# Autodesk Inventor assembly: Shooter Assembly v2
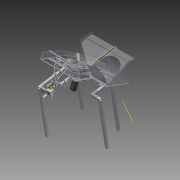
[picture p0: Inventor's stored thumbnail of the model, 180x180]
Saved by Autodesk Inventor 2013 (Build 170138000, 138)
## iProperties
Created: 2013-01-15
Part Number: Shooter Assembly v2
Document SubType Name: Assembly
Designer: actoennies
Mass: 9287.46 g
Surface Area: 30291.7 cm^2
Volume: 4988.3 cm^3
Density: 1.86185 g/cm^3
Author: actoennies
## Documents named in this file (40)
- H:\frc2013CAD-master\Launcher\Shooter\Shooter Assembly v2.iam
- H:\frc2013CAD-master\Launcher\Shooter\Bearing Mount v1.ipt
- H:\frc2013CAD-master\Launcher\Shooter\Outer Rail v1.ipt
- H:\frc2013CAD-master\Launcher\Shooter\Runner Rails v2.ipt
- H:\frc2013CAD-master\Launcher\Shooter\Bearing.ipt
- H:\frc2013CAD-master\Launcher\Shooter\Flywheel Assembly.iam
- H:\frc2013CAD-master\Launcher\Shooter\Shooter Mounter.ipt
- H:\frc2013CAD-master\Launcher\Shooter\Bearing Mount 2 v1.ipt
- H:\frc2013CAD-master\Launcher\Shooter\Shorter Shaft.ipt
- H:\frc2013CAD-master\Launcher\Shooter\Spacer Rube.ipt
- H:\frc2013CAD-master\Launcher\Shooter\Edge Mount.ipt
- H:\frc2013CAD-master\Launcher\Shooter\Square Tube.ipt
- H:\frc2013CAD-master\Launcher\Shooter\Flange Bearing Mount Tower.ipt
- H:\frc2013CAD-master\Launcher\Shooter\Flange Bearing Mount Tower Mirror.ipt
- H:\frc2013CAD-master\Launcher\Shooter\Bearing Mount Top.ipt
- H:\frc2013CAD-master\Launcher\Shooter\Square Motor Mount.ipt
- H:\frc2013CAD-master\Launcher\Shooter\Shooter Assembly v2\Design Accelerator\Spur Gears1.iam
- H:\frc2013CAD-master\Launcher\Parts\Imported Components\Snow Blower Motor\Snow Blower Motor.iam
- H:\frc2013CAD-master\Launcher\Shooter\Snowblower Motor Mount.ipt
- H:\frc2013CAD-master\Launcher\Shooter\8mm shaft.ipt
- H:\frc2013CAD-master\Launcher\Shooter\CIM Bearing.ipt
- H:\frc2013CAD-master\Launcher\Parts\8 Plaction Wheel.iam
- H:\frc2013CAD-master\Launcher\Shooter\Square Tube 2.ipt
- H:\frc2013CAD-master\Launcher\Parts\CIM Motor\Motors_FR801-001.iam
- H:\frc2013CAD-master\Launcher\Shooter\Cim Mount.ipt
- H:\frc2013CAD-master\Launcher\Shooter\Hub v1.ipt
- H:\frc2013CAD-master\Launcher\Shooter\Camera Traffic Light Mount.ipt
- H:\frc2013CAD-master\Launcher\Shooter\Camera Gusset Plat.ipt
- H:\frc2013CAD-master\Launcher\Shooter\Square Tube 3.ipt
- H:\frc2013CAD-master\Launcher\Shooter\edge mount shortened.ipt
- H:\frc2013CAD-master\Launcher\Shooter\Camera.ipt
- H:\frc2013CAD-master\Launcher\Shooter\Square Tube 6.ipt
- H:\frc2013CAD-master\Launcher\Parts\NR-025_5-D(F,D-770).iam
- H:\frc2013CAD-master\Launcher\Shooter\Cylinder Mount.ipt
- H:\frc2013CAD-master\Launcher\Shooter\Cylinder Mount 2.ipt
- H:\frc2013CAD-master\Launcher\Shooter\Gusset Connector.ipt
- H:\frc2013CAD-master\Launcher\Shooter\Gusset Connector 2.ipt
- H:\frc2013CAD-master\Launcher\Shooter\Upper Rails.ipt
- H:\frc2013CAD-master\Launcher\Hopper New\Hopper Assembly.iam
- H:\frc2013CAD-master\Launcher\Hopper New\Puller Mechanism.ipt
## Components (52 placed, 39 different names)
1. Bearing Mount v1:1 — Insert:13, Insert:26, Insert:27, Mate:62, Mate:63, Flush:70, Insert:60, Insert:61, Mate:167
2. Outer Rail v1:1 — Insert:13, Insert:47, Insert:48, Flush:70, Mate:165
3. Runner Rails v2:1 — Insert:60, Insert:61, Mate:166
4. Flywheel Assembly:1 [sub-assembly] — Mate:61, Flush:30, Mate:68, Flush:31
5. Shooter Mounter:1 — Insert:26, Insert:27, Insert:34, Flush:11, Insert:35, Insert:36, Insert:37, Insert:38, Flush:19, Mate:45, Flush:40, Flush:61, Flush:62, Flush:63, Flush:64, Mate:154, Mate:155, Mate:156, Mate:157, Flush:65, Flush:72, Angle:6, Angle:7
6. Spacer Rube:1 — Insert:34, Flush:11
7. Bearing Mount 2 v1:1 — Insert:37, Insert:38, Insert:40
8. Bearing Mount 2 v1:2 — Insert:35, Insert:36, Insert:39
9. Bearing:3 — Insert:40, Flush:13, Mate:14, Mate:15
10. Bearing:4 — Insert:39, Flush:12, Mate:12, Mate:13, Mate:36, Mate:44
11. Shorter Shaft:1 — Flush:12, Mate:12, Mate:13, Mate:37
12. Shorter Shaft:2 — Flush:13, Mate:14, Mate:15, Mate:38
13. Edge Mount:2 — Flush:34, Mate:104, Flush:48, Mate:105, Mate:106, Flush:51, Flush:52, Flush:68
14. Square Tube:2 — Insert:41, Insert:42, Flush:19, Flush:23, Mate:52, Flush:27, Mate:81, Flush:32, Mate:93, Flush:41, Flush:42, Mate:125, Mate:126, Mate:130, Flush:50
15. Flange Bearing Mount Tower:1 — Insert:41, Insert:42, Insert:43
16. Bearing:5 — Insert:43, Mate:36, Mate:37
17. Flange Bearing Mount Tower Mirror:1 — Flush:55, Flush:56, Mate:135, Insert:59
18. Bearing:6 — Mate:38, Insert:59
19. Bearing Mount Top:1 — Insert:47, Insert:48, Mate:65, Mate:66, Mate:68, Mate:162, Mate:163, Mate:164
20. Square Motor Mount:1 — Flush:23, Mate:47, Mate:51, Flush:27, Mate:131
21. Spur Gears:1 [sub-assembly] — Mate:44, Mate:45, Flush:25, Mate:46, Angle:2, Mate:148, Mate:151, Mate:152, Mate:153, Flush:64, Angle:6
22. Snow Blower Motor:1 [sub-assembly] — Flush:25, Mate:46, Angle:2, Insert:50, Insert:51
23. Snowblower Motor Mount:1 — Insert:50, Insert:51, Mate:47, Mate:51, Mate:52
24. 8mm shaft:1 — Mate:61, Flush:30, Mate:67, Flush:31, Mate:82, Mate:83, Mate:84, Mate:86, Mate:167
25. CIM Bearing:1 — Mate:65, Mate:66, Mate:67
26. CIM Bearing:2 — Mate:62, Mate:63, Insert:56
27. 8 Plaction Wheel:1 [sub-assembly] — Mate:88, Mate:89, Mate:90, Mate:91, Mate:92
28. Square Tube 2:1 — Mate:81, Flush:32, Flush:34, Mate:106, Mate:107, Mate:124, Flush:49, Mate:126, Flush:56
29. Motors_FR801-001:1 [sub-assembly] — Mate:82, Mate:83, Mate:84, Mate:143, Mate:144, Mate:145
30. Cim Mount:1 — Flush:40, Mate:143, Mate:144, Mate:145
31. Hub v1:1 — Mate:88, Mate:89, Mate:90, Flush:38
32. Hub v1:2 — Mate:91, Flush:38, Mate:92, Insert:56
33. Camera Traffic Light Mount:1 — Mate:93, Flush:41, Flush:42, Mate:94, Flush:43, Mate:127, Mate:128, Mate:129
34. Camera Gusset Plat:1 — Mate:94, Flush:43, Mate:133
35. Square Tube 3:1 — Mate:104, Flush:48, Mate:105, Mate:107, Mate:132, Flush:55, Mate:135, Mate:146, Flush:58, Flush:59
36. edge mount shortened:1 — Mate:124, Mate:125, Flush:49
37. Camera:1 — Mate:127, Mate:128, Mate:129
38. Edge Mount:3 — Mate:130, Mate:131, Flush:50, Mate:133
39. Edge Mount:4 — Mate:132, Flush:51, Flush:52, Mate:134, Flush:53, Flush:54
40. Square Tube 6:1 — Mate:134, Flush:53, Flush:54, Flush:57, Mate:147, Flush:60
41. NR-025_5-D(F,D-770):1 [sub-assembly] — Mate:136, Mate:137, Mate:138, Mate:139, Mate:140, Insert:62
42. Cylinder Mount:1 — Mate:136, Mate:137, Mate:138, Angle:5
43. Cylinder Mount 2:1 — Mate:139, Mate:140, Angle:5
44. Gusset Connector:1 — Mate:147, Flush:59, Flush:60
45. Gusset Connector:2 — Mate:146, Flush:57, Flush:58
46. Gusset Connector 2:1 — Mate:148, Flush:61, Mate:154
47. Gusset Connector 2:2 — Mate:152, Mate:157, Flush:65
48. Gusset Connector 2:3 — Mate:151, Flush:62, Mate:155
49. Gusset Connector 2:4 — Mate:153, Flush:63, Mate:156
50. Upper Rails:1 — Mate:162, Mate:163, Mate:164
51. Hopper Assembly:1 [sub-assembly] — Flush:72, Mate:165, Mate:166
52. Puller Mechanism:1 — Insert:62, Angle:7
## Relationships (135: Mate 72, Flush 37, Insert 22, Angle 4)
- Insert:13: Bearing Mount v1:1 ↔ Outer Rail v1:1
- Insert:26: Bearing Mount v1:1 ↔ Shooter Mounter:1
- Insert:27: Bearing Mount v1:1 ↔ Shooter Mounter:1
- Insert:34: Shooter Mounter:1 ↔ Spacer Rube:1
- Flush:11: Shooter Mounter:1 ↔ Spacer Rube:1
- Insert:35: Shooter Mounter:1 ↔ Bearing Mount 2 v1:2
- Insert:36: Shooter Mounter:1 ↔ Bearing Mount 2 v1:2
- Insert:37: Shooter Mounter:1 ↔ Bearing Mount 2 v1:1
- Insert:38: Shooter Mounter:1 ↔ Bearing Mount 2 v1:1
- Insert:39: Bearing Mount 2 v1:2 ↔ Bearing:4
- Insert:40: Bearing Mount 2 v1:1 ↔ Bearing:3
- Flush:12 (-25.4 mm): Bearing:4 ↔ Shorter Shaft:1
- Mate:12: Bearing:4 ↔ Shorter Shaft:1
- Mate:13: Bearing:4 ↔ Shorter Shaft:1
- Flush:13 (-25.4 mm): Bearing:3 ↔ Shorter Shaft:2
- Mate:14: Bearing:3 ↔ Shorter Shaft:2
- Mate:15: Bearing:3 ↔ Shorter Shaft:2
- Insert:41: Square Tube:2 ↔ Flange Bearing Mount Tower:1
- Insert:42: Square Tube:2 ↔ Flange Bearing Mount Tower:1
- Insert:43: Flange Bearing Mount Tower:1 ↔ Bearing:5
- Flush:19: Shooter Mounter:1 ↔ Square Tube:2
- Mate:36: Bearing:4 ↔ Bearing:5
- Mate:37: Shorter Shaft:1 ↔ Bearing:5
- Mate:38: Shorter Shaft:2 ↔ Bearing:6
- Insert:47: Outer Rail v1:1 ↔ Bearing Mount Top:1
- Insert:48: Outer Rail v1:1 ↔ Bearing Mount Top:1
- Flush:23 (152.4 mm): Square Tube:2 ↔ Square Motor Mount:1
- Mate:44: Bearing:4 ↔ Spur Gears:1
- Mate:45 (25.4 mm): Shooter Mounter:1 ↔ Spur Gears:1
- Flush:25 (-3.175 mm): Spur Gears:1 ↔ Snow Blower Motor:1
- Mate:46: Spur Gears:1 ↔ Snow Blower Motor:1
- Angle:2 (0 deg): Spur Gears:1 ↔ Snow Blower Motor:1
- Insert:50: Snow Blower Motor:1 ↔ Snowblower Motor Mount:1
- Insert:51: Snow Blower Motor:1 ↔ Snowblower Motor Mount:1
- Mate:47: Square Motor Mount:1 ↔ Snowblower Motor Mount:1
- Mate:51: Square Motor Mount:1 ↔ Snowblower Motor Mount:1
- Mate:52: Square Tube:2 ↔ Snowblower Motor Mount:1
- Flush:27: Square Tube:2 ↔ Square Motor Mount:1
- Mate:61: Flywheel Assembly:1 ↔ 8mm shaft:1
- Flush:30 (12.7 mm): Flywheel Assembly:1 ↔ 8mm shaft:1
- Mate:62: Bearing Mount v1:1 ↔ CIM Bearing:2
- Mate:63: Bearing Mount v1:1 ↔ CIM Bearing:2
- Mate:65: Bearing Mount Top:1 ↔ CIM Bearing:1
- Mate:66: Bearing Mount Top:1 ↔ CIM Bearing:1
- Mate:67: 8mm shaft:1 ↔ CIM Bearing:1
- Mate:68 (6.35 mm): Flywheel Assembly:1 ↔ Bearing Mount Top:1
- Flush:31: Flywheel Assembly:1 ↔ 8mm shaft:1
- Mate:81: Square Tube:2 ↔ Square Tube 2:1
- Flush:32: Square Tube:2 ↔ Square Tube 2:1
- Flush:34: Edge Mount:2 ↔ Square Tube 2:1
- Mate:82: 8mm shaft:1 ↔ Motors_FR801-001:1
- Mate:83: 8mm shaft:1 ↔ Motors_FR801-001:1
- Mate:84: 8mm shaft:1 ↔ Motors_FR801-001:1
- Mate:86: 8mm shaft:1
- Mate:88: 8 Plaction Wheel:1 ↔ Hub v1:1
- Mate:89: 8 Plaction Wheel:1 ↔ Hub v1:1
- Mate:90: 8 Plaction Wheel:1 ↔ Hub v1:1
- Mate:91: 8 Plaction Wheel:1 ↔ Hub v1:2
- Flush:38: Hub v1:1 ↔ Hub v1:2
- Mate:92: 8 Plaction Wheel:1 ↔ Hub v1:2
- Insert:56 (3.175 mm): CIM Bearing:2 ↔ Hub v1:2
- Flush:40: Shooter Mounter:1 ↔ Cim Mount:1
- Mate:93: Square Tube:2 ↔ Camera Traffic Light Mount:1
- Flush:41: Square Tube:2 ↔ Camera Traffic Light Mount:1
- Flush:42: Square Tube:2 ↔ Camera Traffic Light Mount:1
- Mate:94: Camera Traffic Light Mount:1 ↔ Camera Gusset Plat:1
- Flush:43 (11.1125 mm): Camera Traffic Light Mount:1 ↔ Camera Gusset Plat:1
- Mate:104: Edge Mount:2 ↔ Square Tube 3:1
- Flush:48: Edge Mount:2 ↔ Square Tube 3:1
- Mate:105: Edge Mount:2 ↔ Square Tube 3:1
- Mate:106: Edge Mount:2 ↔ Square Tube 2:1
- Mate:107: Square Tube 2:1 ↔ Square Tube 3:1
- Mate:124: Square Tube 2:1 ↔ edge mount shortened:1
- Mate:125: Square Tube:2 ↔ edge mount shortened:1
- Flush:49: Square Tube 2:1 ↔ edge mount shortened:1
- Mate:126: Square Tube:2 ↔ Square Tube 2:1
- Mate:127: Camera Traffic Light Mount:1 ↔ Camera:1
- Mate:128: Camera Traffic Light Mount:1 ↔ Camera:1
- Mate:129: Camera Traffic Light Mount:1 ↔ Camera:1
- Mate:130: Square Tube:2 ↔ Edge Mount:3
- Mate:131: Square Motor Mount:1 ↔ Edge Mount:3
- Flush:50: Square Tube:2 ↔ Edge Mount:3
- Mate:132: Square Tube 3:1 ↔ Edge Mount:4
- Flush:51 (247.65 mm): Edge Mount:2 ↔ Edge Mount:4
- Flush:52 (-95.25 mm): Edge Mount:2 ↔ Edge Mount:4
- Mate:133: Camera Gusset Plat:1 ↔ Edge Mount:3
- Mate:134: Edge Mount:4 ↔ Square Tube 6:1
- Flush:53: Edge Mount:4 ↔ Square Tube 6:1
- Flush:54: Edge Mount:4 ↔ Square Tube 6:1
- Flush:55: Flange Bearing Mount Tower Mirror:1 ↔ Square Tube 3:1
- Flush:56: Flange Bearing Mount Tower Mirror:1 ↔ Square Tube 2:1
- Mate:135: Flange Bearing Mount Tower Mirror:1 ↔ Square Tube 3:1
- Insert:59: Flange Bearing Mount Tower Mirror:1 ↔ Bearing:6
- Mate:136: NR-025_5-D(F,D-770):1 ↔ Cylinder Mount:1
- Mate:137: NR-025_5-D(F,D-770):1 ↔ Cylinder Mount:1
- Mate:138: NR-025_5-D(F,D-770):1 ↔ Cylinder Mount:1
- Mate:139: NR-025_5-D(F,D-770):1 ↔ Cylinder Mount 2:1
- Mate:140: NR-025_5-D(F,D-770):1 ↔ Cylinder Mount 2:1
- Angle:5 (180 deg): Cylinder Mount:1 ↔ Cylinder Mount 2:1
- Mate:143: Motors_FR801-001:1 ↔ Cim Mount:1
- Mate:144: Motors_FR801-001:1 ↔ Cim Mount:1
- Mate:145: Motors_FR801-001:1 ↔ Cim Mount:1
- Mate:146: Square Tube 3:1 ↔ Gusset Connector:2
- Flush:57: Square Tube 6:1 ↔ Gusset Connector:2
- Flush:58: Square Tube 3:1 ↔ Gusset Connector:2
- Mate:147: Square Tube 6:1 ↔ Gusset Connector:1
- Flush:59: Square Tube 3:1 ↔ Gusset Connector:1
- Flush:60: Square Tube 6:1 ↔ Gusset Connector:1
- Mate:148: Spur Gears:1 ↔ Gusset Connector 2:1
- Flush:61 (11.1125 mm): Shooter Mounter:1 ↔ Gusset Connector 2:1
- Mate:151: Spur Gears:1 ↔ Gusset Connector 2:3
- Flush:62 (11.1125 mm): Shooter Mounter:1 ↔ Gusset Connector 2:3
- Mate:152: Spur Gears:1 ↔ Gusset Connector 2:2
- Mate:153: Spur Gears:1 ↔ Gusset Connector 2:4
- Flush:63 (11.1125 mm): Shooter Mounter:1 ↔ Gusset Connector 2:4
- Flush:64 (3.175 mm): Shooter Mounter:1 ↔ Spur Gears:1
- Mate:154: Shooter Mounter:1 ↔ Gusset Connector 2:1
- Mate:155: Shooter Mounter:1 ↔ Gusset Connector 2:3
- Mate:156: Shooter Mounter:1 ↔ Gusset Connector 2:4
- Mate:157: Shooter Mounter:1 ↔ Gusset Connector 2:2
- Flush:65 (11.1125 mm): Shooter Mounter:1 ↔ Gusset Connector 2:2
- Mate:162: Bearing Mount Top:1 ↔ Upper Rails:1
- Mate:163: Bearing Mount Top:1 ↔ Upper Rails:1
- Mate:164: Bearing Mount Top:1 ↔ Upper Rails:1
- Flush:68 (-950.9125 mm): Edge Mount:2
- Flush:70: Bearing Mount v1:1 ↔ Outer Rail v1:1
- Flush:72: Shooter Mounter:1 ↔ Hopper Assembly:1
- Insert:60: Bearing Mount v1:1 ↔ Runner Rails v2:1
- Insert:61: Bearing Mount v1:1 ↔ Runner Rails v2:1
- Mate:165: Outer Rail v1:1 ↔ Hopper Assembly:1
- Mate:166: Runner Rails v2:1 ↔ Hopper Assembly:1
- Angle:6 (180 deg): Shooter Mounter:1 ↔ Spur Gears:1
- Mate:167: Bearing Mount v1:1 ↔ 8mm shaft:1
- Insert:62 (3.175 mm): NR-025_5-D(F,D-770):1 ↔ Puller Mechanism:1
- Angle:7 (180 deg): Shooter Mounter:1 ↔ Puller Mechanism:1
